# Autodesk Inventor assembly: foot2
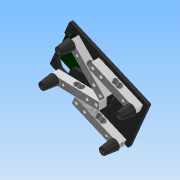
[picture p0: Inventor's stored thumbnail of the model, 180x180]
Saved by Autodesk Inventor 2015 (Build 190159000, 159)
## iProperties
Created: 2015-06-16
Part Number: foot2
Document SubType Name: Assembly
Designer: Gregwar
Author: Gregwar
## Documents named in this file (5)
- C:\Users\Gregwar\Desktop\forcefoot\3d\assembly.iam
- C:\Users\Gregwar\Desktop\forcefoot\3d\foot.ipt
- C:\Users\Gregwar\Desktop\forcefoot\3d\gauge.ipt
- C:\Users\Gregwar\Desktop\forcefoot\3d\cleat.ipt
- C:\Users\Gregwar\Desktop\forcefoot\3d\board.ipt
## Components (10 placed, 4 different names)
1. foot:1 — Placage:1, Placage:2, Placage:3, Placage:4, Placage:5, Placage:6, Placage:7, Placage:8, Placage:9, Placage:10, Placage:11, Placage:12, Placage:21, Placage:22, Placage:23
2. gauge:1 — Placage:1, Placage:2, Placage:3, Placage:17, Placage:18
3. gauge:2 — Placage:7, Placage:8, Placage:9, Placage:15, Placage:16
4. gauge:3 — Placage:4, Placage:5, Placage:6, Placage:13, Placage:14
5. gauge:4 — Placage:10, Placage:11, Placage:12, Placage:19, Placage:20
6. cleat:1 — Placage:13, Placage:14
7. cleat:2 — Placage:17, Placage:18
8. cleat:3 — Placage:19, Placage:20
9. cleat:4 — Placage:15, Placage:16
10. board:1 — Placage:21, Placage:22, Placage:23
## Relationships (23: Mate 23)
- Placage:1 [Mate]: foot:1 ↔ gauge:1
- Placage:2 [Mate]: foot:1 ↔ gauge:1
- Placage:3 [Mate]: foot:1 ↔ gauge:1
- Placage:4 [Mate]: foot:1 ↔ gauge:3
- Placage:5 [Mate]: foot:1 ↔ gauge:3
- Placage:6 [Mate]: foot:1 ↔ gauge:3
- Placage:7 [Mate]: foot:1 ↔ gauge:2
- Placage:8 [Mate]: foot:1 ↔ gauge:2
- Placage:9 [Mate]: foot:1 ↔ gauge:2
- Placage:10 [Mate]: foot:1 ↔ gauge:4
- Placage:11 [Mate]: foot:1 ↔ gauge:4
- Placage:12 [Mate]: foot:1 ↔ gauge:4
- Placage:13 [Mate]: gauge:3 ↔ cleat:1
- Placage:14 [Mate]: gauge:3 ↔ cleat:1
- Placage:15 [Mate]: gauge:2 ↔ cleat:4
- Placage:16 [Mate]: gauge:2 ↔ cleat:4
- Placage:17 [Mate]: gauge:1 ↔ cleat:2
- Placage:18 [Mate]: gauge:1 ↔ cleat:2
- Placage:19 [Mate]: gauge:4 ↔ cleat:3
- Placage:20 [Mate]: gauge:4 ↔ cleat:3
- Placage:21 [Mate]: foot:1 ↔ board:1
- Placage:22 [Mate]: foot:1 ↔ board:1
- Placage:23 [Mate]: foot:1 ↔ board:1
